# Autodesk Inventor assembly: Amante Guisante
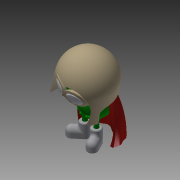
[picture p0: Inventor's stored thumbnail of the model, 180x180]
Saved by Autodesk Inventor 2014 (Build 180170000, 170)
## iProperties
Created: 2015-01-02
Part Number: Amante Guisante
Document SubType Name: Assembly
Designer: Rubén
Author: Rubén
## Documents named in this file (7)
- C:\Users\Rubén\Dropbox\Pendiente\Proyectos\Imprimir\Amante Guisante\Amante Guisante.iam
- C:\Users\Rubén\Dropbox\Pendiente\Proyectos\Imprimir\Amante Guisante\Guisante.ipt
- C:\Users\Rubén\Dropbox\Pendiente\Proyectos\Imprimir\Amante Guisante\Casco.ipt
- C:\Users\Rubén\Dropbox\Pendiente\Proyectos\Imprimir\Amante Guisante\Bota.ipt
- C:\Users\Rubén\Dropbox\Pendiente\Proyectos\Imprimir\Amante Guisante\Capa.ipt
- C:\Users\Rubén\Dropbox\Pendiente\Proyectos\Imprimir\Amante Guisante\Gafas.ipt
- C:\Users\Rubén\Dropbox\Pendiente\Proyectos\Imprimir\Amante Guisante\Ojos.ipt
## Components (7 placed, 6 different names)
1. Guisante:1 — Mate:1, Mate:2, Mate:3, Mate:4, Mate:5, Mate:6, Mate:7, Mate:8, Mate:9, Mate:10, Mate:18, Mate:19, Mate:20, Mate:21, Mate:22, Mate:23
2. Casco:1 — Mate:1, Mate:2, Mate:3
3. Bota:1 — Mate:4, Mate:6
4. Bota:2 — Mate:5, Mate:7
5. Capa:1 — Mate:8, Mate:9, Mate:10
6. Gafas:1 — Mate:18, Mate:19, Mate:20
7. Ojos:1 — Mate:21, Mate:22, Mate:23
## Relationships (16: Mate 16)
- Mate:1: Guisante:1 ↔ Casco:1
- Mate:2: Guisante:1 ↔ Casco:1
- Mate:3 (0.1 mm): Guisante:1 ↔ Casco:1
- Mate:4: Guisante:1 ↔ Bota:1
- Mate:5: Guisante:1 ↔ Bota:2
- Mate:6: Guisante:1 ↔ Bota:1
- Mate:7: Guisante:1 ↔ Bota:2
- Mate:8: Guisante:1 ↔ Capa:1
- Mate:9: Guisante:1 ↔ Capa:1
- Mate:10: Guisante:1 ↔ Capa:1
- Mate:18: Guisante:1 ↔ Gafas:1
- Mate:19: Guisante:1 ↔ Gafas:1
- Mate:20 (0.15 mm): Guisante:1 ↔ Gafas:1
- Mate:21 (0.15 mm): Guisante:1 ↔ Ojos:1
- Mate:22 (0.15 mm): Guisante:1 ↔ Ojos:1
- Mate:23 (1.053 mm): Guisante:1 ↔ Ojos:1
